# Autodesk Inventor assembly: Side cabinet
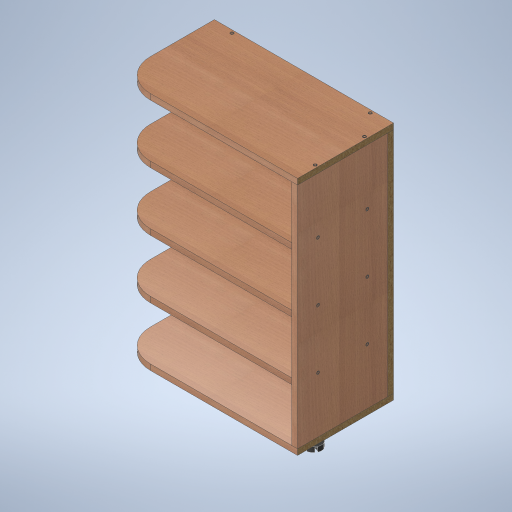
[picture p0: Inventor's stored thumbnail of the model, 512x512]
Saved by Autodesk Inventor 2024 (Build 280153000, 153)
## iProperties
RuleStatus: InUse
Created: 2017-01-19
Part Number: Side cabinet
Document SubType Name: Assembly
Designer: SvetlanaB
Author: SvetlanaB
## Documents named in this file (12)
- C:\W4INV 2024 Design\iBOX LIBRARY\Kitchen\Standing Cabinets\Side cabinet\Side cabinet.iam
- C:\W4INV 2024 Design\iBOX LIBRARY\Kitchen\Standing Cabinets\Side cabinet\Top_panel.ipt
- C:\W4INV 2024 Design\iBOX LIBRARY\Kitchen\Standing Cabinets\Side cabinet\Right_panel.ipt
- C:\W4INV 2024 Design\iBOX LIBRARY\Kitchen\Standing Cabinets\Side cabinet\Bottom_panel.ipt
- C:\W4INV 2024 Design\iBOX LIBRARY\Kitchen\Standing Cabinets\Side cabinet\Back_panel.ipt
- C:\W4INV 2024 Design\iBOX LIBRARY\Kitchen\Standing Cabinets\Side cabinet\Top_panel1.ipt
- C:\W4INV 2024 Design\_LIBRARY\Supports and legs\Legs\ADJUSTABLE LEG\Adjustable leg  BT18 clip included.ipt
- C:\W4INV 2024 Design\iBOX LIBRARY\Kitchen\Standing Cabinets\Side cabinet\Shelf.ipt
- C:\W4INV 2024 Design\iBOX LIBRARY\Kitchen\Standing Cabinets\Side cabinet\Side cabinet.ipt
- C:\W4INV 2024 Design\_LIBRARY\Fixed joints\Confirmat\CONFIRMAT\Confirmat L50 NB T18 PB T 18.ipt
- C:\W4INV 2023 Design\LIBRARY\Fixed joints\Confirmat\CONFIRMAT.ipt
- C:\W4INV 2023 Design\LIBRARY\Supports and legs\Legs\ADJUSTABLE LEG.ipt
## Components (31 placed, 9 different names)
1. @Skeleton
2. Top_panel:1 — Nestled Board Plane:5, Nestled Board Plane:6, Nestled Board Plane:9, Nestled Board Plane:11
3. Right_panel:1 — Flush:1, Flush:4, Flush:5, Pillar Board Side Plane:1, Pillar Board Side Plane:2, Nestled Board Plane:7, Nestled Board Plane:8, Pillar Board Side Plane:9, Pillar Board Side Plane:11
4. Bottom_panel:1 — Flush:2, Flush:3, Bottom board Plane:1, Bottom board Plane:2, Front (Angle) Plane:1, Front (Angle) Plane:2, Nestled Board Plane:1, Nestled Board Plane:2, Nestled Board Plane:3, Nestled Board Plane:4
5. Back_panel:1 — Flush:6, Flush:7, Pillar Board Side Plane:3, Pillar Board Side Plane:4, Nestled Board Plane:10, Nestled Board Plane:12, Pillar Board Side Plane:5, Pillar Board Side Plane:6
6. Top_panel1:1
7. Adjustable leg  BT18 clip included:1 — Bottom board Plane:1, Axis Plane:1, Axis2 Plane:1, Front (Angle) Plane:2
8. Adjustable leg  BT18 clip included:2 — Bottom board Plane:2, Axis Plane:2, Axis2 Plane:2, Front (Angle) Plane:1
9. Confirmat L50 NB T18 PB T 18:1 — Axis Plane:3, Nestled Board Plane:1, Pillar Board Side Plane:1
10. Confirmat L50 NB T18 PB T 18:2 — Axis Plane:4, Nestled Board Plane:2, Pillar Board Side Plane:2
11. Confirmat L50 NB T18 PB T 18:3 — Axis Plane:5, Nestled Board Plane:3, Pillar Board Side Plane:3
12. Confirmat L50 NB T18 PB T 18:4 — Axis Plane:6, Nestled Board Plane:4, Pillar Board Side Plane:4
13. Confirmat L50 NB T18 PB T 18:22 — Nestled Board Plane:5, Pillar Board Side Plane:5, Axis Plane:7
14. Confirmat L50 NB T18 PB T 18:23 — Nestled Board Plane:6, Pillar Board Side Plane:6, Axis Plane:8
15. Confirmat L50 NB T18 PB T 18:24 — Nestled Board Plane:9, Pillar Board Side Plane:9, Axis Plane:11
16. Confirmat L50 NB T18 PB T 18:25 — Nestled Board Plane:11, Pillar Board Side Plane:11, Axis Plane:13
17. Shelf:1 — Pillar Board Side Plane:7, Pillar Board Side Plane:8, Pillar Board Side Plane:10, Pillar Board Side Plane:12
18. Confirmat L50 NB T18 PB T 18:9 — Axis Plane:10, Nestled Board Plane:8, Pillar Board Side Plane:8
19. Confirmat L50 NB T18 PB T 18:8 — Axis Plane:9, Nestled Board Plane:7, Pillar Board Side Plane:7
20. Confirmat L50 NB T18 PB T 18:13 — Axis Plane:14, Pillar Board Side Plane:12, Nestled Board Plane:12
21. Confirmat L50 NB T18 PB T 18:11 — Axis Plane:12, Pillar Board Side Plane:10, Nestled Board Plane:10
22. Shelf:2
23. Confirmat L50 NB T18 PB T 18:14
24. Confirmat L50 NB T18 PB T 18:16
25. Confirmat L50 NB T18 PB T 18:18
26. Confirmat L50 NB T18 PB T 18:20
27. Shelf:3
28. Confirmat L50 NB T18 PB T 18:15
29. Confirmat L50 NB T18 PB T 18:17
30. Confirmat L50 NB T18 PB T 18:19
31. Confirmat L50 NB T18 PB T 18:21
## Component patterns: (3 elements, first: Shelf:1 + Confirmat L50 NB T18 PB T 18:9 + Confirmat L50 NB T18 PB T 18:8 + Confirmat L50 NB T18 PB T 18:13 + Confirmat L50 NB T18 PB T 18:11)
## Relationships (51: Mate 30, Flush 19, Angle 2)
- Flush:1 (-100 mm): Right_panel:1
- Flush:2 (-100 mm): Bottom_panel:1
- Flush:3 (-150 mm): Bottom_panel:1
- Bottom board Plane:1 [Mate]: Bottom_panel:1 ↔ Adjustable leg  BT18 clip included:1
- Axis Plane:1 [Mate]: Adjustable leg  BT18 clip included:1
- Axis2 Plane:1 [Mate]: Adjustable leg  BT18 clip included:1
- Bottom board Plane:2 [Mate]: Bottom_panel:1 ↔ Adjustable leg  BT18 clip included:2
- Axis Plane:2 [Mate]: Adjustable leg  BT18 clip included:2
- Axis2 Plane:2 [Mate]: Adjustable leg  BT18 clip included:2
- Flush:4 (-64 mm): Right_panel:1
- Flush:5 (-64 mm): Right_panel:1
- Flush:6 (-64 mm): Back_panel:1
- Flush:7 (-64 mm): Back_panel:1
- Front (Angle) Plane:1 [Angle] (0 deg): Bottom_panel:1 ↔ Adjustable leg  BT18 clip included:2
- Front (Angle) Plane:2 [Angle] (0 deg): Bottom_panel:1 ↔ Adjustable leg  BT18 clip included:1
- Axis Plane:3 [Mate]: Confirmat L50 NB T18 PB T 18:1
- Nestled Board Plane:1 [Flush]: Bottom_panel:1 ↔ Confirmat L50 NB T18 PB T 18:1
- Pillar Board Side Plane:1 [Mate] (-9 mm): Right_panel:1 ↔ Confirmat L50 NB T18 PB T 18:1
- Axis Plane:4 [Mate]: Confirmat L50 NB T18 PB T 18:2
- Nestled Board Plane:2 [Flush]: Bottom_panel:1 ↔ Confirmat L50 NB T18 PB T 18:2
- Pillar Board Side Plane:2 [Mate] (-9 mm): Right_panel:1 ↔ Confirmat L50 NB T18 PB T 18:2
- Axis Plane:5 [Mate]: Confirmat L50 NB T18 PB T 18:3
- Nestled Board Plane:3 [Flush]: Bottom_panel:1 ↔ Confirmat L50 NB T18 PB T 18:3
- Pillar Board Side Plane:3 [Mate] (-9 mm): Back_panel:1 ↔ Confirmat L50 NB T18 PB T 18:3
- Axis Plane:6 [Mate]: Confirmat L50 NB T18 PB T 18:4
- Nestled Board Plane:4 [Flush]: Bottom_panel:1 ↔ Confirmat L50 NB T18 PB T 18:4
- Pillar Board Side Plane:4 [Mate] (-9 mm): Back_panel:1 ↔ Confirmat L50 NB T18 PB T 18:4
- Axis Plane:9 [Mate]: Confirmat L50 NB T18 PB T 18:8
- Nestled Board Plane:7 [Flush]: Right_panel:1 ↔ Confirmat L50 NB T18 PB T 18:8
- Pillar Board Side Plane:7 [Mate] (-9 mm): Shelf:1 ↔ Confirmat L50 NB T18 PB T 18:8
- Axis Plane:10 [Mate]: Confirmat L50 NB T18 PB T 18:9
- Nestled Board Plane:8 [Flush]: Right_panel:1 ↔ Confirmat L50 NB T18 PB T 18:9
- Pillar Board Side Plane:8 [Mate] (-9 mm): Shelf:1 ↔ Confirmat L50 NB T18 PB T 18:9
- Axis Plane:12 [Mate]: Confirmat L50 NB T18 PB T 18:11
- Pillar Board Side Plane:10 [Mate] (-9 mm): Shelf:1 ↔ Confirmat L50 NB T18 PB T 18:11
- Nestled Board Plane:10 [Flush]: Back_panel:1 ↔ Confirmat L50 NB T18 PB T 18:11
- Axis Plane:14 [Mate]: Confirmat L50 NB T18 PB T 18:13
- Pillar Board Side Plane:12 [Mate] (-9 mm): Shelf:1 ↔ Confirmat L50 NB T18 PB T 18:13
- Nestled Board Plane:12 [Flush]: Back_panel:1 ↔ Confirmat L50 NB T18 PB T 18:13
- Nestled Board Plane:5 [Flush]: Top_panel:1 ↔ Confirmat L50 NB T18 PB T 18:22
- Pillar Board Side Plane:5 [Mate] (-9 mm): Back_panel:1 ↔ Confirmat L50 NB T18 PB T 18:22
- Axis Plane:7 [Mate]: Confirmat L50 NB T18 PB T 18:22
- Nestled Board Plane:6 [Flush]: Top_panel:1 ↔ Confirmat L50 NB T18 PB T 18:23
- Pillar Board Side Plane:6 [Mate] (-9 mm): Back_panel:1 ↔ Confirmat L50 NB T18 PB T 18:23
- Axis Plane:8 [Mate]: Confirmat L50 NB T18 PB T 18:23
- Nestled Board Plane:9 [Flush]: Top_panel:1 ↔ Confirmat L50 NB T18 PB T 18:24
- Pillar Board Side Plane:9 [Mate] (-9 mm): Right_panel:1 ↔ Confirmat L50 NB T18 PB T 18:24
- Axis Plane:11 [Mate]: Confirmat L50 NB T18 PB T 18:24
- Nestled Board Plane:11 [Flush]: Top_panel:1 ↔ Confirmat L50 NB T18 PB T 18:25
- Pillar Board Side Plane:11 [Mate] (-9 mm): Right_panel:1 ↔ Confirmat L50 NB T18 PB T 18:25
- Axis Plane:13 [Mate]: Confirmat L50 NB T18 PB T 18:25
## Named parameters: Shelf_quantity = 3, Panel_thickness = 18 mm, Distance_between_shelfs = 165 mm
